# Autodesk Inventor assembly: Montagem1
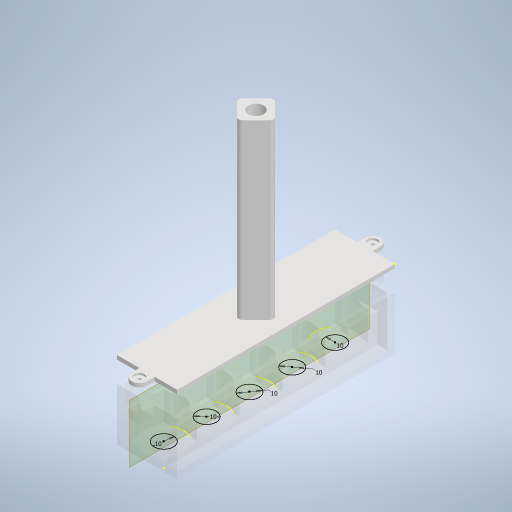
[picture p0: Inventor's stored thumbnail of the model, 512x512]
Saved by Autodesk Inventor 2023 (Build 270158000, 158)
## iProperties
Created: 2023-03-29
Part Number: Montagem1
Document SubType Name: Assembly
Designer: Inteli
Author: Inteli
## Documents named in this file (3)
- C:\Users\Inteli\Documents\GitHub\grupo5\docs\desenhos_tecnicos\modelo_3D\Montagem1.iam
- C:\Users\Inteli\Documents\GitHub\grupo5\docs\desenhos_tecnicos\modelo_3D\Suporte 4 EletroImã.ipt
- C:\Users\Inteli\Documents\GitHub\grupo5\docs\desenhos_tecnicos\modelo_3D\Tampa Suporte 4E.ipt
## Components (2 placed, 2 different names)
1. Suporte 4 EletroImã:1 — Coincidente:1, Coincidente:2
2. Tampa Suporte 4E:1 — Coincidente:1, Coincidente:2
## Relationships (2: Mate 2)
- Coincidente:1 [Mate]: Suporte 4 EletroImã:1 ↔ Tampa Suporte 4E:1
- Coincidente:2 [Mate]: Suporte 4 EletroImã:1 ↔ Tampa Suporte 4E:1
